# Autodesk Inventor assembly: MainAssembly
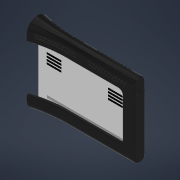
[picture p0: Inventor's stored thumbnail of the model, 180x180]
Saved by Autodesk Inventor 2022 (Build 260153000, 153)
## iProperties
Created: 2021-08-31
Part Number: MainAssembly
Document SubType Name: Assembly
Designer: trl121
Author: trl121
## Documents named in this file (6)
- D:\trl121\Documents\_repositories\RazerBook13Dock\Inventor\MainAssembly.iam
- D:\trl121\Documents\_repositories\RazerBook13Dock\Inventor\Razor Book 13.ipt
- D:\trl121\Documents\_repositories\RazerBook13Dock\Inventor\BottomPart.ipt
- D:\trl121\Documents\_repositories\RazerBook13Dock\Inventor\UpperPart.ipt
- D:\trl121\Documents\_repositories\RazerBook13Dock\Inventor\Mount_.ipt
- D:\trl121\Documents\_repositories\RazerBook13Dock\Inventor\USBCClamp.ipt
## Components (6 placed, 5 different names)
1. Razor Book 13:1 — Flush:1, Flush:2, Mate:1, Flush:4
2. BottomPart:1 — Flush:3, Flush:4, Flush:5, Flush:6, Flush:8, Flush:10, Mate:7, Mate:8, Insert:1, Flush:12
3. UpperPart:1 — Flush:7, Mate:2, Flush:8, Mate:6, Mate:9
4. Mount_:1 — Flush:9, Mate:4, Mate:5, Flush:10, Mate:9
5. Mount_:2 — Mate:7, Mate:8, Insert:1
6. USBCClamp:1 — Flush:11, Mate:10, Mate:11, Flush:12
## Relationships (23: Flush 12, Mate 10, Insert 1)
- Flush:1: Razor Book 13:1
- Flush:2: Razor Book 13:1
- Mate:1: Razor Book 13:1
- Flush:3: BottomPart:1
- Flush:4: Razor Book 13:1 ↔ BottomPart:1
- Flush:5: BottomPart:1
- Flush:6: BottomPart:1
- Flush:7: UpperPart:1
- Mate:2: UpperPart:1
- Flush:8: BottomPart:1 ↔ UpperPart:1
- Flush:9: Mount_:1
- Mate:4: Mount_:1
- Mate:5: Mount_:1
- Flush:10 (0.1016 mm): BottomPart:1 ↔ Mount_:1
- Mate:6: UpperPart:1
- Mate:7: BottomPart:1 ↔ Mount_:2
- Mate:8 (0.2 mm): BottomPart:1 ↔ Mount_:2
- Insert:1: BottomPart:1 ↔ Mount_:2
- Mate:9: UpperPart:1 ↔ Mount_:1
- Flush:11: USBCClamp:1
- Mate:10: USBCClamp:1
- Mate:11: USBCClamp:1
- Flush:12: BottomPart:1 ↔ USBCClamp:1
